# Autodesk Inventor assembly: DesignRootModel^PCB_ESP32-C3-MINI-1_V1(2)_PCB_ESP32-C3-MINI-1_V1
(part 2 of 2)
- C:\Users\test\Projects\WearableWLED\WearableWLED_Mechanical\board\WearableWLED_Hardware\WearableWLED_Hardware\uid__1-253^DesignRootModel_PCB_ESP32-C3-MINI-1_V1(2)_PCB_ESP32-C3-MINI-1_V1.ipt
- C:\Users\test\Projects\WearableWLED\WearableWLED_Mechanical\board\WearableWLED_Hardware\WearableWLED_Hardware\uid__1-254^DesignRootModel_PCB_ESP32-C3-MINI-1_V1(2)_PCB_ESP32-C3-MINI-1_V1.ipt
- C:\Users\test\Projects\WearableWLED\WearableWLED_Mechanical\board\WearableWLED_Hardware\WearableWLED_Hardware\uid__1-255^DesignRootModel_PCB_ESP32-C3-MINI-1_V1(2)_PCB_ESP32-C3-MINI-1_V1.ipt
- C:\Users\test\Projects\WearableWLED\WearableWLED_Mechanical\board\WearableWLED_Hardware\WearableWLED_Hardware\uid__1-256^DesignRootModel_PCB_ESP32-C3-MINI-1_V1(2)_PCB_ESP32-C3-MINI-1_V1.ipt
- C:\Users\test\Projects\WearableWLED\WearableWLED_Mechanical\board\WearableWLED_Hardware\WearableWLED_Hardware\uid__1-257^DesignRootModel_PCB_ESP32-C3-MINI-1_V1(2)_PCB_ESP32-C3-MINI-1_V1.ipt
- C:\Users\test\Projects\WearableWLED\WearableWLED_Mechanical\board\WearableWLED_Hardware\WearableWLED_Hardware\uid__1-258^DesignRootModel_PCB_ESP32-C3-MINI-1_V1(2)_PCB_ESP32-C3-MINI-1_V1.ipt
- C:\Users\test\Projects\WearableWLED\WearableWLED_Mechanical\board\WearableWLED_Hardware\WearableWLED_Hardware\uid__1-259^DesignRootModel_PCB_ESP32-C3-MINI-1_V1(2)_PCB_ESP32-C3-MINI-1_V1.ipt
- C:\Users\test\Projects\WearableWLED\WearableWLED_Mechanical\board\WearableWLED_Hardware\WearableWLED_Hardware\uid__1-260^DesignRootModel_PCB_ESP32-C3-MINI-1_V1(2)_PCB_ESP32-C3-MINI-1_V1.ipt
- C:\Users\test\Projects\WearableWLED\WearableWLED_Mechanical\board\WearableWLED_Hardware\WearableWLED_Hardware\uid__1-261^DesignRootModel_PCB_ESP32-C3-MINI-1_V1(2)_PCB_ESP32-C3-MINI-1_V1.ipt
- C:\Users\test\Projects\WearableWLED\WearableWLED_Mechanical\board\WearableWLED_Hardware\WearableWLED_Hardware\uid__1-262^DesignRootModel_PCB_ESP32-C3-MINI-1_V1(2)_PCB_ESP32-C3-MINI-1_V1.ipt
- C:\Users\test\Projects\WearableWLED\WearableWLED_Mechanical\board\WearableWLED_Hardware\WearableWLED_Hardware\uid__1-263^DesignRootModel_PCB_ESP32-C3-MINI-1_V1(2)_PCB_ESP32-C3-MINI-1_V1.ipt
- C:\Users\test\Projects\WearableWLED\WearableWLED_Mechanical\board\WearableWLED_Hardware\WearableWLED_Hardware\uid__1-264^DesignRootModel_PCB_ESP32-C3-MINI-1_V1(2)_PCB_ESP32-C3-MINI-1_V1.ipt
- C:\Users\test\Projects\WearableWLED\WearableWLED_Mechanical\board\WearableWLED_Hardware\WearableWLED_Hardware\uid__1-265^DesignRootModel_PCB_ESP32-C3-MINI-1_V1(2)_PCB_ESP32-C3-MINI-1_V1.ipt
- C:\Users\test\Projects\WearableWLED\WearableWLED_Mechanical\board\WearableWLED_Hardware\WearableWLED_Hardware\uid__1-266^DesignRootModel_PCB_ESP32-C3-MINI-1_V1(2)_PCB_ESP32-C3-MINI-1_V1.ipt
- C:\Users\test\Projects\WearableWLED\WearableWLED_Mechanical\board\WearableWLED_Hardware\WearableWLED_Hardware\uid__1-267^DesignRootModel_PCB_ESP32-C3-MINI-1_V1(2)_PCB_ESP32-C3-MINI-1_V1.ipt
- C:\Users\test\Projects\WearableWLED\WearableWLED_Mechanical\board\WearableWLED_Hardware\WearableWLED_Hardware\uid__1-268^DesignRootModel_PCB_ESP32-C3-MINI-1_V1(2)_PCB_ESP32-C3-MINI-1_V1.ipt
- C:\Users\test\Projects\WearableWLED\WearableWLED_Mechanical\board\WearableWLED_Hardware\WearableWLED_Hardware\uid__1-269^DesignRootModel_PCB_ESP32-C3-MINI-1_V1(2)_PCB_ESP32-C3-MINI-1_V1.ipt
- C:\Users\test\Projects\WearableWLED\WearableWLED_Mechanical\board\WearableWLED_Hardware\WearableWLED_Hardware\uid__1-270^DesignRootModel_PCB_ESP32-C3-MINI-1_V1(2)_PCB_ESP32-C3-MINI-1_V1.ipt
- C:\Users\test\Projects\WearableWLED\WearableWLED_Mechanical\board\WearableWLED_Hardware\WearableWLED_Hardware\uid__1-271^DesignRootModel_PCB_ESP32-C3-MINI-1_V1(2)_PCB_ESP32-C3-MINI-1_V1.ipt
- C:\Users\test\Projects\WearableWLED\WearableWLED_Mechanical\board\WearableWLED_Hardware\WearableWLED_Hardware\uid__1-272^DesignRootModel_PCB_ESP32-C3-MINI-1_V1(2)_PCB_ESP32-C3-MINI-1_V1.ipt
- C:\Users\test\Projects\WearableWLED\WearableWLED_Mechanical\board\WearableWLED_Hardware\WearableWLED_Hardware\uid__1-273^DesignRootModel_PCB_ESP32-C3-MINI-1_V1(2)_PCB_ESP32-C3-MINI-1_V1.ipt
- C:\Users\test\Projects\WearableWLED\WearableWLED_Mechanical\board\WearableWLED_Hardware\WearableWLED_Hardware\uid__1-274^DesignRootModel_PCB_ESP32-C3-MINI-1_V1(2)_PCB_ESP32-C3-MINI-1_V1.ipt
- C:\Users\test\Projects\WearableWLED\WearableWLED_Mechanical\board\WearableWLED_Hardware\WearableWLED_Hardware\uid__1-275^DesignRootModel_PCB_ESP32-C3-MINI-1_V1(2)_PCB_ESP32-C3-MINI-1_V1.ipt
- C:\Users\test\Projects\WearableWLED\WearableWLED_Mechanical\board\WearableWLED_Hardware\WearableWLED_Hardware\uid__1-276^DesignRootModel_PCB_ESP32-C3-MINI-1_V1(2)_PCB_ESP32-C3-MINI-1_V1.ipt
- C:\Users\test\Projects\WearableWLED\WearableWLED_Mechanical\board\WearableWLED_Hardware\WearableWLED_Hardware\uid__1-277^DesignRootModel_PCB_ESP32-C3-MINI-1_V1(2)_PCB_ESP32-C3-MINI-1_V1.ipt
- C:\Users\test\Projects\WearableWLED\WearableWLED_Mechanical\board\WearableWLED_Hardware\WearableWLED_Hardware\uid__1-278^DesignRootModel_PCB_ESP32-C3-MINI-1_V1(2)_PCB_ESP32-C3-MINI-1_V1.ipt
- C:\Users\test\Projects\WearableWLED\WearableWLED_Mechanical\board\WearableWLED_Hardware\WearableWLED_Hardware\uid__1-279^DesignRootModel_PCB_ESP32-C3-MINI-1_V1(2)_PCB_ESP32-C3-MINI-1_V1.ipt
- C:\Users\test\Projects\WearableWLED\WearableWLED_Mechanical\board\WearableWLED_Hardware\WearableWLED_Hardware\uid__1-280^DesignRootModel_PCB_ESP32-C3-MINI-1_V1(2)_PCB_ESP32-C3-MINI-1_V1.ipt
- C:\Users\test\Projects\WearableWLED\WearableWLED_Mechanical\board\WearableWLED_Hardware\WearableWLED_Hardware\uid__1-281^DesignRootModel_PCB_ESP32-C3-MINI-1_V1(2)_PCB_ESP32-C3-MINI-1_V1.ipt
- C:\Users\test\Projects\WearableWLED\WearableWLED_Mechanical\board\WearableWLED_Hardware\WearableWLED_Hardware\uid__1-282^DesignRootModel_PCB_ESP32-C3-MINI-1_V1(2)_PCB_ESP32-C3-MINI-1_V1.ipt
- C:\Users\test\Projects\WearableWLED\WearableWLED_Mechanical\board\WearableWLED_Hardware\WearableWLED_Hardware\uid__1-283^DesignRootModel_PCB_ESP32-C3-MINI-1_V1(2)_PCB_ESP32-C3-MINI-1_V1.ipt
- C:\Users\test\Projects\WearableWLED\WearableWLED_Mechanical\board\WearableWLED_Hardware\WearableWLED_Hardware\uid__1-284^DesignRootModel_PCB_ESP32-C3-MINI-1_V1(2)_PCB_ESP32-C3-MINI-1_V1.ipt
- C:\Users\test\Projects\WearableWLED\WearableWLED_Mechanical\board\WearableWLED_Hardware\WearableWLED_Hardware\uid__1-285^DesignRootModel_PCB_ESP32-C3-MINI-1_V1(2)_PCB_ESP32-C3-MINI-1_V1.ipt
- C:\Users\test\Projects\WearableWLED\WearableWLED_Mechanical\board\WearableWLED_Hardware\WearableWLED_Hardware\uid__1-286^DesignRootModel_PCB_ESP32-C3-MINI-1_V1(2)_PCB_ESP32-C3-MINI-1_V1.ipt
- C:\Users\test\Projects\WearableWLED\WearableWLED_Mechanical\board\WearableWLED_Hardware\WearableWLED_Hardware\uid__1-287^DesignRootModel_PCB_ESP32-C3-MINI-1_V1(2)_PCB_ESP32-C3-MINI-1_V1.ipt
- C:\Users\test\Projects\WearableWLED\WearableWLED_Mechanical\board\WearableWLED_Hardware\WearableWLED_Hardware\uid__1-288^DesignRootModel_PCB_ESP32-C3-MINI-1_V1(2)_PCB_ESP32-C3-MINI-1_V1.ipt
- C:\Users\test\Projects\WearableWLED\WearableWLED_Mechanical\board\WearableWLED_Hardware\WearableWLED_Hardware\uid__1-289^DesignRootModel_PCB_ESP32-C3-MINI-1_V1(2)_PCB_ESP32-C3-MINI-1_V1.ipt
- C:\Users\test\Projects\WearableWLED\WearableWLED_Mechanical\board\WearableWLED_Hardware\WearableWLED_Hardware\uid__1-290^DesignRootModel_PCB_ESP32-C3-MINI-1_V1(2)_PCB_ESP32-C3-MINI-1_V1.ipt
- C:\Users\test\Projects\WearableWLED\WearableWLED_Mechanical\board\WearableWLED_Hardware\WearableWLED_Hardware\uid__1-291^DesignRootModel_PCB_ESP32-C3-MINI-1_V1(2)_PCB_ESP32-C3-MINI-1_V1.ipt
- C:\Users\test\Projects\WearableWLED\WearableWLED_Mechanical\board\WearableWLED_Hardware\WearableWLED_Hardware\uid__1-292^DesignRootModel_PCB_ESP32-C3-MINI-1_V1(2)_PCB_ESP32-C3-MINI-1_V1.ipt
- C:\Users\test\Projects\WearableWLED\WearableWLED_Mechanical\board\WearableWLED_Hardware\WearableWLED_Hardware\uid__1-293^DesignRootModel_PCB_ESP32-C3-MINI-1_V1(2)_PCB_ESP32-C3-MINI-1_V1.ipt
- C:\Users\test\Projects\WearableWLED\WearableWLED_Mechanical\board\WearableWLED_Hardware\WearableWLED_Hardware\uid__1-294^DesignRootModel_PCB_ESP32-C3-MINI-1_V1(2)_PCB_ESP32-C3-MINI-1_V1.ipt
- C:\Users\test\Projects\WearableWLED\WearableWLED_Mechanical\board\WearableWLED_Hardware\WearableWLED_Hardware\uid__1-295^DesignRootModel_PCB_ESP32-C3-MINI-1_V1(2)_PCB_ESP32-C3-MINI-1_V1.ipt
- C:\Users\test\Projects\WearableWLED\WearableWLED_Mechanical\board\WearableWLED_Hardware\WearableWLED_Hardware\uid__1-296^DesignRootModel_PCB_ESP32-C3-MINI-1_V1(2)_PCB_ESP32-C3-MINI-1_V1.ipt
- C:\Users\test\Projects\WearableWLED\WearableWLED_Mechanical\board\WearableWLED_Hardware\WearableWLED_Hardware\uid__1-297^DesignRootModel_PCB_ESP32-C3-MINI-1_V1(2)_PCB_ESP32-C3-MINI-1_V1.ipt
- C:\Users\test\Projects\WearableWLED\WearableWLED_Mechanical\board\WearableWLED_Hardware\WearableWLED_Hardware\uid__1-298^DesignRootModel_PCB_ESP32-C3-MINI-1_V1(2)_PCB_ESP32-C3-MINI-1_V1.ipt
- C:\Users\test\Projects\WearableWLED\WearableWLED_Mechanical\board\WearableWLED_Hardware\WearableWLED_Hardware\uid__1-299^DesignRootModel_PCB_ESP32-C3-MINI-1_V1(2)_PCB_ESP32-C3-MINI-1_V1.ipt
- C:\Users\test\Projects\WearableWLED\WearableWLED_Mechanical\board\WearableWLED_Hardware\WearableWLED_Hardware\uid__1-300^DesignRootModel_PCB_ESP32-C3-MINI-1_V1(2)_PCB_ESP32-C3-MINI-1_V1.ipt
- C:\Users\test\Projects\WearableWLED\WearableWLED_Mechanical\board\WearableWLED_Hardware\WearableWLED_Hardware\uid__1-301^DesignRootModel_PCB_ESP32-C3-MINI-1_V1(2)_PCB_ESP32-C3-MINI-1_V1.ipt
- C:\Users\test\Projects\WearableWLED\WearableWLED_Mechanical\board\WearableWLED_Hardware\WearableWLED_Hardware\uid__1-302^DesignRootModel_PCB_ESP32-C3-MINI-1_V1(2)_PCB_ESP32-C3-MINI-1_V1.ipt
- C:\Users\test\Projects\WearableWLED\WearableWLED_Mechanical\board\WearableWLED_Hardware\WearableWLED_Hardware\uid__1-303^DesignRootModel_PCB_ESP32-C3-MINI-1_V1(2)_PCB_ESP32-C3-MINI-1_V1.ipt
- C:\Users\test\Projects\WearableWLED\WearableWLED_Mechanical\board\WearableWLED_Hardware\WearableWLED_Hardware\uid__1-304^DesignRootModel_PCB_ESP32-C3-MINI-1_V1(2)_PCB_ESP32-C3-MINI-1_V1.ipt
- C:\Users\test\Projects\WearableWLED\WearableWLED_Mechanical\board\WearableWLED_Hardware\WearableWLED_Hardware\uid__1-305^DesignRootModel_PCB_ESP32-C3-MINI-1_V1(2)_PCB_ESP32-C3-MINI-1_V1.ipt
- C:\Users\test\Projects\WearableWLED\WearableWLED_Mechanical\board\WearableWLED_Hardware\WearableWLED_Hardware\uid__1-306^DesignRootModel_PCB_ESP32-C3-MINI-1_V1(2)_PCB_ESP32-C3-MINI-1_V1.ipt
- C:\Users\test\Projects\WearableWLED\WearableWLED_Mechanical\board\WearableWLED_Hardware\WearableWLED_Hardware\uid__1-307^DesignRootModel_PCB_ESP32-C3-MINI-1_V1(2)_PCB_ESP32-C3-MINI-1_V1.ipt
- C:\Users\test\Projects\WearableWLED\WearableWLED_Mechanical\board\WearableWLED_Hardware\WearableWLED_Hardware\uid__1-308^DesignRootModel_PCB_ESP32-C3-MINI-1_V1(2)_PCB_ESP32-C3-MINI-1_V1.ipt
- C:\Users\test\Projects\WearableWLED\WearableWLED_Mechanical\board\WearableWLED_Hardware\WearableWLED_Hardware\uid__1-309^DesignRootModel_PCB_ESP32-C3-MINI-1_V1(2)_PCB_ESP32-C3-MINI-1_V1.ipt
- C:\Users\test\Projects\WearableWLED\WearableWLED_Mechanical\board\WearableWLED_Hardware\WearableWLED_Hardware\uid__1-310^DesignRootModel_PCB_ESP32-C3-MINI-1_V1(2)_PCB_ESP32-C3-MINI-1_V1.ipt
- C:\Users\test\Projects\WearableWLED\WearableWLED_Mechanical\board\WearableWLED_Hardware\WearableWLED_Hardware\uid__1-311^DesignRootModel_PCB_ESP32-C3-MINI-1_V1(2)_PCB_ESP32-C3-MINI-1_V1.ipt
- C:\Users\test\Projects\WearableWLED\WearableWLED_Mechanical\board\WearableWLED_Hardware\WearableWLED_Hardware\uid__1-312^DesignRootModel_PCB_ESP32-C3-MINI-1_V1(2)_PCB_ESP32-C3-MINI-1_V1.ipt
- C:\Users\test\Projects\WearableWLED\WearableWLED_Mechanical\board\WearableWLED_Hardware\WearableWLED_Hardware\uid__1-313^DesignRootModel_PCB_ESP32-C3-MINI-1_V1(2)_PCB_ESP32-C3-MINI-1_V1.ipt
- C:\Users\test\Projects\WearableWLED\WearableWLED_Mechanical\board\WearableWLED_Hardware\WearableWLED_Hardware\uid__1-314^DesignRootModel_PCB_ESP32-C3-MINI-1_V1(2)_PCB_ESP32-C3-MINI-1_V1.ipt
- C:\Users\test\Projects\WearableWLED\WearableWLED_Mechanical\board\WearableWLED_Hardware\WearableWLED_Hardware\uid__1-315^DesignRootModel_PCB_ESP32-C3-MINI-1_V1(2)_PCB_ESP32-C3-MINI-1_V1.ipt
- C:\Users\test\Projects\WearableWLED\WearableWLED_Mechanical\board\WearableWLED_Hardware\WearableWLED_Hardware\uid__1-316^DesignRootModel_PCB_ESP32-C3-MINI-1_V1(2)_PCB_ESP32-C3-MINI-1_V1.ipt
- C:\Users\test\Projects\WearableWLED\WearableWLED_Mechanical\board\WearableWLED_Hardware\WearableWLED_Hardware\uid__1-317^DesignRootModel_PCB_ESP32-C3-MINI-1_V1(2)_PCB_ESP32-C3-MINI-1_V1.ipt
- C:\Users\test\Projects\WearableWLED\WearableWLED_Mechanical\board\WearableWLED_Hardware\WearableWLED_Hardware\uid__1-318^DesignRootModel_PCB_ESP32-C3-MINI-1_V1(2)_PCB_ESP32-C3-MINI-1_V1.ipt
- C:\Users\test\Projects\WearableWLED\WearableWLED_Mechanical\board\WearableWLED_Hardware\WearableWLED_Hardware\uid__1-319^DesignRootModel_PCB_ESP32-C3-MINI-1_V1(2)_PCB_ESP32-C3-MINI-1_V1.ipt
- C:\Users\test\Projects\WearableWLED\WearableWLED_Mechanical\board\WearableWLED_Hardware\WearableWLED_Hardware\uid__1-320^DesignRootModel_PCB_ESP32-C3-MINI-1_V1(2)_PCB_ESP32-C3-MINI-1_V1.ipt
- C:\Users\test\Projects\WearableWLED\WearableWLED_Mechanical\board\WearableWLED_Hardware\WearableWLED_Hardware\uid__1-321^DesignRootModel_PCB_ESP32-C3-MINI-1_V1(2)_PCB_ESP32-C3-MINI-1_V1.ipt
- C:\Users\test\Projects\WearableWLED\WearableWLED_Mechanical\board\WearableWLED_Hardware\WearableWLED_Hardware\uid__1-322^DesignRootModel_PCB_ESP32-C3-MINI-1_V1(2)_PCB_ESP32-C3-MINI-1_V1.ipt
- C:\Users\test\Projects\WearableWLED\WearableWLED_Mechanical\board\WearableWLED_Hardware\WearableWLED_Hardware\uid__1-323^DesignRootModel_PCB_ESP32-C3-MINI-1_V1(2)_PCB_ESP32-C3-MINI-1_V1.ipt
- C:\Users\test\Projects\WearableWLED\WearableWLED_Mechanical\board\WearableWLED_Hardware\WearableWLED_Hardware\uid__1-324^DesignRootModel_PCB_ESP32-C3-MINI-1_V1(2)_PCB_ESP32-C3-MINI-1_V1.ipt
- C:\Users\test\Projects\WearableWLED\WearableWLED_Mechanical\board\WearableWLED_Hardware\WearableWLED_Hardware\uid__1-325^DesignRootModel_PCB_ESP32-C3-MINI-1_V1(2)_PCB_ESP32-C3-MINI-1_V1.ipt
- C:\Users\test\Projects\WearableWLED\WearableWLED_Mechanical\board\WearableWLED_Hardware\WearableWLED_Hardware\uid__1-326^DesignRootModel_PCB_ESP32-C3-MINI-1_V1(2)_PCB_ESP32-C3-MINI-1_V1.ipt
- C:\Users\test\Projects\WearableWLED\WearableWLED_Mechanical\board\WearableWLED_Hardware\WearableWLED_Hardware\uid__1-327^DesignRootModel_PCB_ESP32-C3-MINI-1_V1(2)_PCB_ESP32-C3-MINI-1_V1.ipt
- C:\Users\test\Projects\WearableWLED\WearableWLED_Mechanical\board\WearableWLED_Hardware\WearableWLED_Hardware\uid__1-328^DesignRootModel_PCB_ESP32-C3-MINI-1_V1(2)_PCB_ESP32-C3-MINI-1_V1.ipt
- C:\Users\test\Projects\WearableWLED\WearableWLED_Mechanical\board\WearableWLED_Hardware\WearableWLED_Hardware\uid__1-329^DesignRootModel_PCB_ESP32-C3-MINI-1_V1(2)_PCB_ESP32-C3-MINI-1_V1.ipt
- C:\Users\test\Projects\WearableWLED\WearableWLED_Mechanical\board\WearableWLED_Hardware\WearableWLED_Hardware\uid__2428^DesignRootModel_PCB_ESP32-C3-MINI-1_V1(2)_PCB_ESP32-C3-MINI-1_V1.ipt
## Components (332 placed, 332 different names)
1. 3 [sub-assembly]
2. 6 [sub-assembly]
3. 17 [sub-assembly]
4. 20 [sub-assembly]
5. 23 [sub-assembly]
6. 26 [sub-assembly]
7. 29 [sub-assembly]
8. 32 [sub-assembly]
9. 35 [sub-assembly]
10. 38 [sub-assembly]
11. 41 [sub-assembly]
12. 44 [sub-assembly]
13. 47 [sub-assembly]
14. 50 [sub-assembly]
15. 53 [sub-assembly]
16. 56 [sub-assembly]
17. 59 [sub-assembly]
18. 62 [sub-assembly]
19. 65 [sub-assembly]
20. 68 [sub-assembly]
21. 71 [sub-assembly]
22. 72
23. 73
24. 74
25. 75
26. 76
27. 77
28. 78
29. 79
30. 80
31. 81
32. 82
33. 83
34. 84
35. 85
36. 86
37. 87
38. 88
39. 89
40. 90
41. 91
42. 92
43. 93
44. 94
45. 95
46. 96
47. 97
48. 98
49. 99
50. 100
51. 101
52. 102
53. 103
54. 104
55. 105
56. 106
57. 107
58. 108
59. 109
60. 110
61. 111
62. 112
63. 113
64. 114
65. 115
66. 116
67. 117
68. 118
69. 119
70. 120
71. 121
72. 122
73. 123
74. 124
75. 125
76. 126
77. 127
78. 128
79. 129
80. 130
81. 131
82. 132
83. 133
84. 134
85. 135
86. 136
87. 137
88. 138
89. 139
90. 140
91. 141
92. 142
93. 143
94. 144
95. 145
96. 146
97. 147
98. 148
99. 149
100. 150
101. 151
102. 152
103. 153
104. 154
105. 155
106. 156
107. 157
108. 158
109. 159
110. 160
111. 161
112. 162
113. 163
114. 164
115. 165
116. 166
117. 167
118. 168
119. 169
120. 170
121. 171
122. 172
123. 173
124. 174
125. 175
126. 176
127. 177
128. 178
129. 179
130. 180
131. 181
132. 182
133. 183
134. 184
135. 185
136. 186
137. 187
138. 188
139. 189
140. 190
141. 191
142. 192
143. 193
144. 194
145. 195
146. 196
147. 197
148. 198
149. 199
150. 200
151. 201
152. 202
153. 203
154. 204
155. 205
156. 206
157. 207
158. 208
159. 209
160. 210
161. 211
162. 212
163. 213
164. 214
165. 215
166. 216
167. 217
168. 218
169. 219
170. 220
171. 221
172. 222
173. 223
174. 224
175. 225
176. 226
177. 227
178. 228
179. 229
180. 230
181. 231
182. 232
183. 233
184. 234
185. 235
186. 236
187. 237
188. 238
189. 239
190. 240
191. 241
192. 242
193. 243
194. 244
195. 245
196. 246
197. 247
198. 248
199. 249
200. 250
201. 251
202. 252
203. 253
204. 254
205. 255
206. 256
207. 257
208. 258
209. 259
210. 260
211. 261
212. 262
213. 263
214. 264
215. 265
216. 266
217. 267
218. 268
219. 269
220. 270
221. 271
222. 272
223. 273
224. 274
225. 275
226. 276
227. 277
228. 278
229. 279
230. 280
231. 281
232. 282
233. 283
234. 284
235. 285
236. 286
237. 287
238. 288
239. 289
240. 290
241. 291
242. 292
243. 293
244. 294
245. 295
246. 296
247. 297
248. 298
249. 299
250. 300
251. 301
252. 302
253. 303
254. 304
255. 305
256. 306
257. 307
258. 308
259. 309
260. 310
261. 311
262. 312
263. 313
264. 314
265. 315
266. 316
267. 317
268. 318
269. 319
270. 320
271. 321
272. 322
273. 323
274. 324
275. 325
276. 326
277. 327
278. 328
279. 329
280. 330
281. 331
282. 332
283. 333
284. 334
285. 335
286. 336
287. 337
288. 338
289. 339
290. 340
291. 341
292. 342
293. 343
294. 344
295. 345
296. 346
297. 347
298. 348
299. 349
300. 350
301. 351
302. 352
303. 353
304. 354
305. 355
306. 356
307. 357
308. 358
309. 359
310. 360
311. 361
312. 362
313. 363
314. 364
315. 365
316. 366
317. 367
318. 368
319. 369
320. 370
321. 371
322. 372
323. 373
324. 374
325. 375
326. 376
327. 377
328. 378
329. 379
330. 380
331. 381
332. 382
